# Autodesk Inventor assembly: Molde_levelled_new
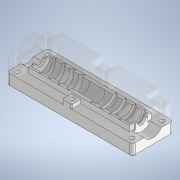
[picture p0: Inventor's stored thumbnail of the model, 180x180]
Saved by Autodesk Inventor 2020 (Build 240168000, 168)
## iProperties
Created: 2021-06-17
Part Number: Molde_levelled_new
Document SubType Name: Assembly
Designer: Acer
Author: Acer
## Documents named in this file (3)
- G:\Meu Drive\RobôCIn\Mecânica\SSL\2021\Inventor\first_floor\Dribbler-3-gears\Molde_levelled_new.iam
- G:\Meu Drive\RobôCIn\Mecânica\SSL\2021\Inventor\first_floor\Dribbler-3-gears\MoldeA_leveled_new.ipt
- G:\Meu Drive\RobôCIn\Mecânica\SSL\2021\Inventor\first_floor\Dribbler-3-gears\MoldeB_leveled_new.ipt
## Components (2 placed, 1 different names)
1. Dribblerschnecke:1 — Mate:1, Mate:2, Mate:3
2. Dribblerschnecke:2 — Mate:1, Mate:2, Mate:3
## Relationships (3: Mate 3)
- Mate:1: Dribblerschnecke:1 ↔ Dribblerschnecke:2
- Mate:2: Dribblerschnecke:1 ↔ Dribblerschnecke:2
- Mate:3: Dribblerschnecke:1 ↔ Dribblerschnecke:2
